# Autodesk Inventor assembly: Full Chassis - Full Assembly
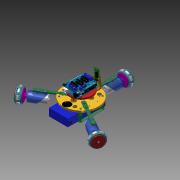
[picture p0: Inventor's stored thumbnail of the model, 180x180]
Saved by Autodesk Inventor 2014 (Build 180170000, 170)
## iProperties
Created: 2014-02-26
Part Number: Full Chassis - Full Assembly
Document SubType Name: Assembly
Designer: Spooner
Author: Spooner
## Documents named in this file (3)
- C:\Users\Spooner\Documents\Inventor\FerretBall Robot\3Pod\Inventor 2014 Files\Full Chassis - Full Assembly.iam
- C:\Users\Spooner\Documents\Inventor\FerretBall Robot\3Pod\Inventor 2014 Files\Main Body - Full Assembly.iam
- C:\Users\Spooner\Documents\Inventor\FerretBall Robot\3Pod\Inventor 2014 Files\Full Motor Arm (1 inch) with Kornylak Wheel.iam
## Components (4 placed, 2 different names)
1. Main Body - Full Assembly:1 [sub-assembly] — Insert:1, Mate:1, Insert:2, Mate:2, Insert:3, Mate:3
2. Full Motor Arm (1 inch) with Kornylak Wheel:1 [sub-assembly] — Insert:3, Mate:3
3. Full Motor Arm (1 inch) with Kornylak Wheel:2 [sub-assembly] — Insert:2, Mate:2
4. Full Motor Arm (1 inch) with Kornylak Wheel:3 [sub-assembly] — Insert:1, Mate:1
## Relationships (6: Insert 3, Mate 3)
- Insert:1: Main Body - Full Assembly:1 ↔ Full Motor Arm (1 inch) with Kornylak Wheel:3
- Mate:1: Main Body - Full Assembly:1 ↔ Full Motor Arm (1 inch) with Kornylak Wheel:3
- Insert:2: Main Body - Full Assembly:1 ↔ Full Motor Arm (1 inch) with Kornylak Wheel:2
- Mate:2: Main Body - Full Assembly:1 ↔ Full Motor Arm (1 inch) with Kornylak Wheel:2
- Insert:3: Main Body - Full Assembly:1 ↔ Full Motor Arm (1 inch) with Kornylak Wheel:1
- Mate:3: Main Body - Full Assembly:1 ↔ Full Motor Arm (1 inch) with Kornylak Wheel:1
